# Autodesk Inventor assembly: mesoSPIM_PI_L-509_Assembly_Draft_V1
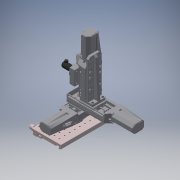
[picture p0: Inventor's stored thumbnail of the model, 180x180]
Saved by Autodesk Inventor 2016 (Build 200138000, 138)
## iProperties
Created: 2018-09-28
Part Number: mesoSPIM_PI_L-509_Assembly_Draft_V1
Document SubType Name: Assembly
Designer: voigt
Author: voigt
## Documents named in this file (8)
- D:\Microscope_Design\CAD_Files\mesoSPIM_design\mesoSPIM\sample_stages\mesoSPIM_PI_L-509_Assembly_Draft_V1.iam
- D:\Microscope_Design\CAD_Files\mesoSPIM_design\library\Qioptiq\X95_carriers\X95_300mm_carrier\X95_300mm_Carrier.iam
- D:\Microscope_Design\CAD_Files\mesoSPIM_design\library\Physik_Instrumente\L-509.20DG10.ipt
- D:\Microscope_Design\CAD_Files\mesoSPIM_design\library\Physik_Instrumente\L-509.40DG10.ipt
- D:\Microscope_Design\CAD_Files\mesoSPIM_design\library\Physik_Instrumente\KUM_L-500.AV3.ipt
- D:\Microscope_Design\CAD_Files\mesoSPIM_design\library\Physik_Instrumente\M-060.DG_KUNDENMODELL.ipt
- D:\Microscope_Design\CAD_Files\mesoSPIM_design\mesoSPIM\sample_stages\M-060-Adapter.ipt
- D:\Microscope_Design\CAD_Files\mesoSPIM_design\library\Thorlabs\posts\post_mounts\PH50_M-Step.ipt
## Components (8 placed, 7 different names)
1. X95_300mm_Carrier:1 [sub-assembly] — Mate:1, Mate:16, Mate:17
2. L-509.20DG10:1 — Mate:1, Mate:2, Mate:3, Mate:4, Mate:16, Mate:17
3. L-509.40DG10:1 — Mate:2, Mate:3, Mate:4, Mate:5, Mate:6, Mate:7
4. KUM_L-500.AV3:1 — Mate:5, Mate:6, Mate:7, Mate:8, Mate:9, Mate:10
5. L-509.20DG10:2 — Mate:8, Mate:9, Mate:10, Mate:18, Mate:19, Mate:20
6. M-060.DG_KUNDENMODELL:1 — Mate:11, Mate:12, Mate:13, Mate:18, Mate:19, Mate:20
7. M-060-Adapter:1 — Mate:11, Mate:12, Mate:13, Mate:14, Mate:15
8. PH50_M-Step:1 — Mate:14, Mate:15
## Relationships (20: Mate 20)
- Mate:1: X95_300mm_Carrier:1 ↔ L-509.20DG10:1
- Mate:2: L-509.20DG10:1 ↔ L-509.40DG10:1
- Mate:3: L-509.20DG10:1 ↔ L-509.40DG10:1
- Mate:4: L-509.20DG10:1 ↔ L-509.40DG10:1
- Mate:5: L-509.40DG10:1 ↔ KUM_L-500.AV3:1
- Mate:6: L-509.40DG10:1 ↔ KUM_L-500.AV3:1
- Mate:7: L-509.40DG10:1 ↔ KUM_L-500.AV3:1
- Mate:8: KUM_L-500.AV3:1 ↔ L-509.20DG10:2
- Mate:9: KUM_L-500.AV3:1 ↔ L-509.20DG10:2
- Mate:10: KUM_L-500.AV3:1 ↔ L-509.20DG10:2
- Mate:11: M-060.DG_KUNDENMODELL:1 ↔ M-060-Adapter:1
- Mate:12: M-060.DG_KUNDENMODELL:1 ↔ M-060-Adapter:1
- Mate:13: M-060.DG_KUNDENMODELL:1 ↔ M-060-Adapter:1
- Mate:14: M-060-Adapter:1 ↔ PH50_M-Step:1
- Mate:15: M-060-Adapter:1 ↔ PH50_M-Step:1
- Mate:16: X95_300mm_Carrier:1 ↔ L-509.20DG10:1
- Mate:17: X95_300mm_Carrier:1 ↔ L-509.20DG10:1
- Mate:18: L-509.20DG10:2 ↔ M-060.DG_KUNDENMODELL:1
- Mate:19: L-509.20DG10:2 ↔ M-060.DG_KUNDENMODELL:1
- Mate:20 (19 mm): L-509.20DG10:2 ↔ M-060.DG_KUNDENMODELL:1
